# Autodesk Inventor assembly: KB33-046-009 - Колпак лидара
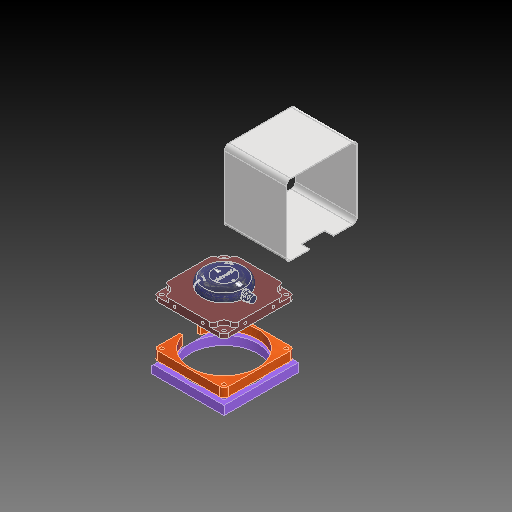
[picture p0: Inventor's stored thumbnail of the model, 512x512]
Saved by Autodesk Inventor 2020 (Build 240168000, 168)
## iProperties
Created: 2021-08-10
Part Number: KB33-046-009 - Колпак лидара
Document SubType Name: Assembly
Designer: Петров Иван
Mass: 133.789 g
Surface Area: 862.526 cm^2
Volume: 133.789 cm^3
Density: 1 g/cm^3
Author: Петров Иван
## Documents named in this file (6)
- E:\IVAN\Ivan_desktop\Kvantorium\Projects\RoboPatrol\design\KB33-046-009 - Колпак лидара.iam
- E:\IVAN\Ivan_desktop\Kvantorium\Projects\RoboPatrol\design\KB33-046-009-001 - Крышка.ipt
- E:\IVAN\Ivan_desktop\Kvantorium\Projects\RoboPatrol\design\standart_components\GPS\PX4 Neo M8N GPS.ipt
- E:\IVAN\Ivan_desktop\Kvantorium\Projects\RoboPatrol\design\KB33-046-009-002 - Прижим верхний.ipt
- E:\IVAN\Ivan_desktop\Kvantorium\Projects\RoboPatrol\design\KB33-046-009-003 - Прижим нижний.ipt
- E:\IVAN\Ivan_desktop\Kvantorium\Projects\RoboPatrol\design\KB33-046-009-004  - Стенка.ipt
## Components (5 placed, 5 different names)
1. KB33-046-009-001 - Крышка:1 — Совмещение:1, Совмещение:2, Угол:1, Совмещение:3, Совмещение:4, Совмещение:5, Совмещение:6
2. PX4 Neo M8N GPS:1 — Совмещение:1, Совмещение:2, Угол:1
3. KB33-046-009-002 - Прижим верхний:1 — Совмещение:3, Совмещение:4, Совмещение:5, Совмещение:7, Совмещение:8
4. KB33-046-009-003 - Прижим нижний:1 — Совмещение:6, Совмещение:7, Совмещение:8, Заподлицо:1
5. KB33-046-009-004  - Стенка:1 — Заподлицо:1
## Relationships (10: Mate 8, Angle 1, Flush 1)
- Совмещение:1 [Mate]: KB33-046-009-001 - Крышка:1 ↔ PX4 Neo M8N GPS:1
- Совмещение:2 [Mate]: KB33-046-009-001 - Крышка:1 ↔ PX4 Neo M8N GPS:1
- Угол:1 [Angle] (0 deg): KB33-046-009-001 - Крышка:1 ↔ PX4 Neo M8N GPS:1
- Совмещение:3 [Mate] (48 mm): KB33-046-009-001 - Крышка:1 ↔ KB33-046-009-002 - Прижим верхний:1
- Совмещение:4 [Mate]: KB33-046-009-001 - Крышка:1 ↔ KB33-046-009-002 - Прижим верхний:1
- Совмещение:5 [Mate]: KB33-046-009-001 - Крышка:1 ↔ KB33-046-009-002 - Прижим верхний:1
- Совмещение:6 [Mate]: KB33-046-009-001 - Крышка:1 ↔ KB33-046-009-003 - Прижим нижний:1
- Совмещение:7 [Mate]: KB33-046-009-002 - Прижим верхний:1 ↔ KB33-046-009-003 - Прижим нижний:1
- Совмещение:8 [Mate] (4 mm): KB33-046-009-002 - Прижим верхний:1 ↔ KB33-046-009-003 - Прижим нижний:1
- Заподлицо:1 [Flush]: KB33-046-009-003 - Прижим нижний:1 ↔ KB33-046-009-004  - Стенка:1
